# Autodesk Inventor assembly: DrillCompleta
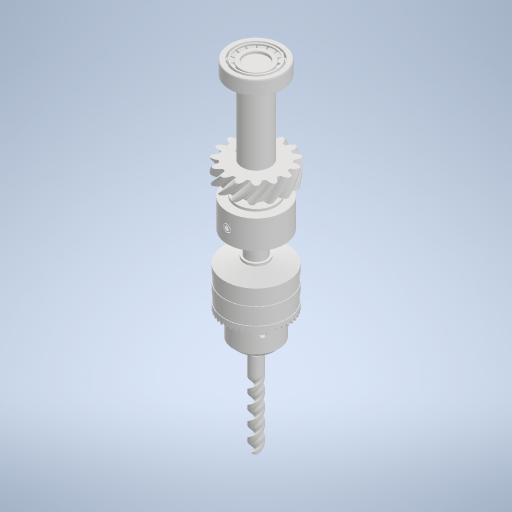
[picture p0: Inventor's stored thumbnail of the model, 512x512]
Saved by Autodesk Inventor 2024.2 (Build 282272000, 272)
## iProperties
Created: 2024-04-19
Part Number: DrillCompleta
Document SubType Name: Assembly
Designer: 062210026
Author: 062210026
## Documents named in this file (3)
- Z:\ProjInt3\Ferramenta\DrillCompleta.iam
- Z:\ProjInt3\Ferramenta\Drill3.ipt
- Z:\ProjInt3\Ferramenta\Escalonada1.ipt
## Components (2 placed, 2 different names)
1. Drill3:1 — Mate:1
2. Escalonada1:1 — Mate:1
## Relationships (1: Mate 1)
- Mate:1: Drill3:1 ↔ Escalonada1:1
